# Autodesk Inventor assembly: Assembly1
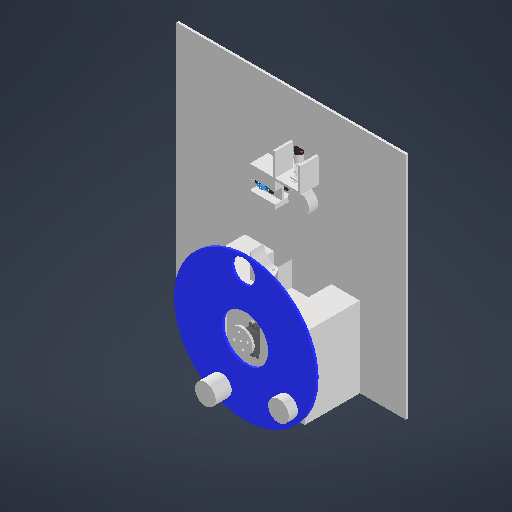
[picture p0: Inventor's stored thumbnail of the model, 512x512]
Saved by Autodesk Inventor 2027.1 (Build 311270010, 270A)
## iProperties
Created: 2026-09-28
Part Number: Assembly1
Document SubType Name: Assembly
Designer: daniel
Author: daniel
## Documents named in this file (11)
- C:\Users\danda\Desktop\Design 1\Project\CAD\Assembly1.iam
- C:\Users\danda\Desktop\Design 1\Project\CAD\Part2.ipt
- C:\Users\danda\Desktop\Design 1\Project\CAD\Part1.ipt
- C:\Users\danda\Desktop\Design 1\Project\CAD\Part3.ipt
- C:\Users\danda\Desktop\Design 1\Project\CAD\base.ipt
- C:\Users\danda\Downloads\standard-servo-motor-black-1.snapshot.7\Assem1\Assem1.iam
- C:\Users\danda\Desktop\Design 1\Project\CAD\Part22.ipt
- C:\Users\danda\Desktop\Design 1\Project\CAD\Part23.ipt
- C:\Users\danda\Desktop\Design 1\Project\CAD\Part24.ipt
- C:\Users\danda\Desktop\Design 1\Project\CAD\Assembly7.iam
- C:\Users\danda\Desktop\Design 1\Project\CAD\Part27.ipt
## Components (10 placed, 10 different names)
1. Part2:1 — Mate:10, Tangent:1, Tangent:2, Mate:18
2. Part1:1 — Mate:8, Mate:9, Mate:10, Mate:11, Mate:15, Mate:16, Mate:17
3. Part3:1 — Mate:3, Mate:4, Mate:6, Mate:7, Flush:2, Flush:3, Mate:11, Mate:20, Flush:22, Flush:23, Flush:24
4. base:1 — Mate:6, Flush:2, Flush:3, Mate:19, Flush:21
5. Assem1:1 [sub-assembly] — Mate:3, Mate:4, Mate:7, Mate:17, Mate:18
6. Part22:1 — Mate:8, Mate:9, Tangent:3, Flush:23, Flush:24
7. Part23:1 — Tangent:1, Mate:15
8. Part24:1 — Mate:16, Tangent:2
9. Assembly7:1 [sub-assembly] — Mate:19, Flush:21
10. Part27:1 — Mate:20, Tangent:3, Flush:22
## Relationships (23: Mate 14, Flush 6, Tangent 3)
- Mate:3: Part3:1 ↔ Assem1:1
- Mate:4: Part3:1 ↔ Assem1:1
- Mate:6: Part3:1 ↔ base:1
- Mate:7: Part3:1 ↔ Assem1:1
- Flush:2 (100 mm): Part3:1 ↔ base:1
- Mate:8: Part1:1 ↔ Part22:1
- Mate:9: Part1:1 ↔ Part22:1
- Flush:3: Part3:1 ↔ base:1
- Mate:10: Part2:1 ↔ Part1:1
- Mate:11: Part1:1 ↔ Part3:1
- Tangent:1: Part2:1 ↔ Part23:1
- Mate:15: Part1:1 ↔ Part23:1
- Mate:16: Part1:1 ↔ Part24:1
- Tangent:2: Part2:1 ↔ Part24:1
- Mate:17: Part1:1 ↔ Assem1:1
- Mate:18: Part2:1 ↔ Assem1:1
- Mate:19: base:1 ↔ Assembly7:1
- Flush:21 (190 mm): base:1 ↔ Assembly7:1
- Mate:20: Part3:1 ↔ Part27:1
- Tangent:3: Part22:1 ↔ Part27:1
- Flush:22: Part3:1 ↔ Part27:1
- Flush:23: Part3:1 ↔ Part22:1
- Flush:24: Part3:1 ↔ Part22:1
